# Autodesk Inventor assembly: Zespół1
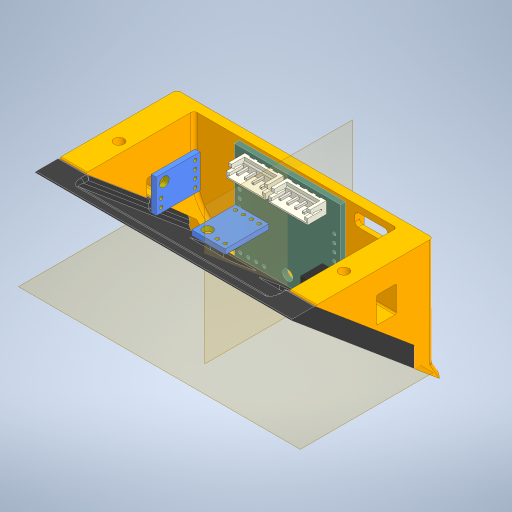
[picture p0: Inventor's stored thumbnail of the model, 512x512]
Saved by Autodesk Inventor 2023 (Build 270158000, 158)
## iProperties
Created: 2024-05-14
Part Number: Zespół1
Document SubType Name: Assembly
Designer: kamil
Author: kamil
## Documents named in this file (5)
- C:\Users\kamil\Documents\PROJECTS - repos\ModBot---Projekt-Zespolowy\mechanics\Zespół1.iam
- C:\Users\kamil\Documents\PROJECTS - repos\ModBot---Projekt-Zespolowy\mechanics\STEP\Moduł Sumo.ipt
- C:\Users\kamil\Documents\PROJECTS - repos\ModBot---Projekt-Zespolowy\mechanics\MS_podstawa.ipt
- C:\Users\kamil\Documents\PROJECTS - repos\ModBot---Projekt-Zespolowy\mechanics\MS_Pokrywa.ipt
- C:\Users\kamil\Documents\PROJECTS - repos\ModBot---Projekt-Zespolowy\mechanics\TOF_VL53L0X (1).ipt
## Components (6 placed, 4 different names)
1. Moduł Sumo:1 — Równoległe:1, Zestawiające:7, Zestawiające:8, Zestawiające:9, Zestawiające:10, Kątowe:1, Kątowe:2, Zestawiające:11, Zestawiające:12, Zestawiające:13, Kątowe:3, Zestawiające:14
2. MS_podstawa:1 — Zestawiające:4, Zestawiające:5, Zestawiające:6, Równoległe:1, Zestawiające:7, Zestawiające:8
3. MS_Pokrywa:1 — Zestawiające:4, Zestawiające:5, Zestawiające:6
4. TOF_VL53L0X (1):1 — Zestawiające:9, Kątowe:1, Zestawiające:11
5. TOF_VL53L0X (1):2 — Zestawiające:10, Kątowe:2, Zestawiające:12
6. TOF_VL53L0X (1):3 — Zestawiające:13, Kątowe:3, Zestawiające:14
## Relationships (15: Mate 11, Angle 3, Flush 1)
- Zestawiające:4 [Mate]: MS_podstawa:1 ↔ MS_Pokrywa:1
- Zestawiające:5 [Mate]: MS_podstawa:1 ↔ MS_Pokrywa:1
- Zestawiające:6 [Mate]: MS_podstawa:1 ↔ MS_Pokrywa:1
- Równoległe:1 [Flush]: Moduł Sumo:1 ↔ MS_podstawa:1
- Zestawiające:7 [Mate] (15.5 mm): Moduł Sumo:1 ↔ MS_podstawa:1
- Zestawiające:8 [Mate] (1 mm): Moduł Sumo:1 ↔ MS_podstawa:1
- Zestawiające:9 [Mate]: Moduł Sumo:1 ↔ TOF_VL53L0X (1):1
- Zestawiające:10 [Mate]: Moduł Sumo:1 ↔ TOF_VL53L0X (1):2
- Kątowe:1 [Angle] (180 deg): Moduł Sumo:1 ↔ TOF_VL53L0X (1):1
- Kątowe:2 [Angle] (180 deg): Moduł Sumo:1 ↔ TOF_VL53L0X (1):2
- Zestawiające:11 [Mate] (-9.4 mm): Moduł Sumo:1 ↔ TOF_VL53L0X (1):1
- Zestawiające:12 [Mate] (-1.9 mm): Moduł Sumo:1 ↔ TOF_VL53L0X (1):2
- Zestawiające:13 [Mate]: Moduł Sumo:1 ↔ TOF_VL53L0X (1):3
- Kątowe:3 [Angle] (180 deg): Moduł Sumo:1 ↔ TOF_VL53L0X (1):3
- Zestawiające:14 [Mate] (-9.4 mm): Moduł Sumo:1 ↔ TOF_VL53L0X (1):3
